# Autodesk Inventor assembly: 8 inch mecanum with toughbox ( Bottom Right)
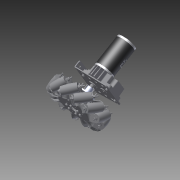
[picture p0: Inventor's stored thumbnail of the model, 180x180]
Saved by Autodesk Inventor 2014 (Build 180170000, 170)
## iProperties
Created: 2015-01-10
Part Number: 8 inch mecanum with toughbox ( Bottom Right)
Document SubType Name: Assembly
Designer: student
Author: student
## Documents named in this file (6)
- C:\Users\student\Documents\Inventor\2015 Recycle Rush\8 inch mecanum with toughbox ( Bottom Right).iam
- C:\Users\student\Documents\Inventor\Dillon And Justin\Derived Right Mecanum_MIR.ipt
- C:\Users\student\Documents\Inventor\2015 Recycle Rush\am-0077a-500 Key Hub r2.ipt
- C:\Users\student\Documents\Inventor\2015 Recycle Rush\Derived Toughbox mini.ipt
- C:\Users\student\Documents\Inventor\Dillon And Justin\Imported Components\MOT_CIM-Motor_217-2000.iam\MOT_CIM-Motor_217-2000.iam.iam
- MOT_CIM-Motor_217-2000.iam
## Components (4 placed, 4 different names)
1. Derived Right Mecanum_MIR:1 — Angle:1, Mate:1, Mate:2, Mate:3, Mate:4
2. am-0077a-500 Key Hub r2:1 — Angle:1, Mate:1, Mate:2, Mate:3, Mate:5
3. Derived Toughbox mini:1 — Mate:4, Mate:5, Angle:2, Angle:3, Mate:6
4. MOT_CIM-Motor_217-2000.iam:1 [sub-assembly] — Angle:3, Mate:6
## Relationships (9: Mate 6, Angle 3)
- Angle:1 (180 deg): Derived Right Mecanum_MIR:1 ↔ am-0077a-500 Key Hub r2:1
- Mate:1: Derived Right Mecanum_MIR:1 ↔ am-0077a-500 Key Hub r2:1
- Mate:2: Derived Right Mecanum_MIR:1 ↔ am-0077a-500 Key Hub r2:1
- Mate:3: Derived Right Mecanum_MIR:1 ↔ am-0077a-500 Key Hub r2:1
- Mate:4: Derived Right Mecanum_MIR:1 ↔ Derived Toughbox mini:1
- Mate:5: am-0077a-500 Key Hub r2:1 ↔ Derived Toughbox mini:1
- Angle:2 (180 deg): Derived Toughbox mini:1
- Angle:3 (180 deg): Derived Toughbox mini:1 ↔ MOT_CIM-Motor_217-2000.iam:1
- Mate:6: Derived Toughbox mini:1 ↔ MOT_CIM-Motor_217-2000.iam:1
